# Autodesk Inventor assembly: ScreenHolderASM
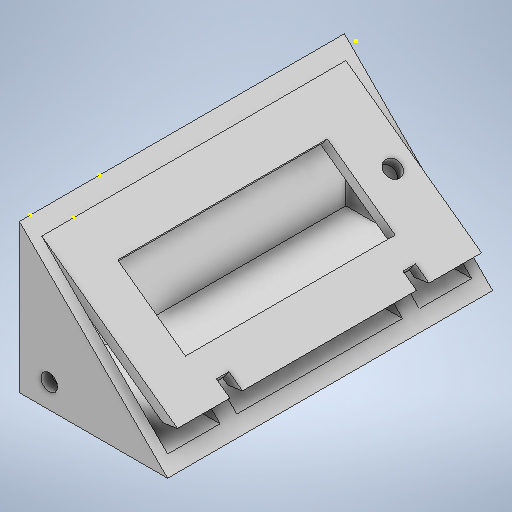
[picture p0: Inventor's stored thumbnail of the model, 512x512]
Saved by Autodesk Inventor 2025 (Build 290162000, 162)
## iProperties
Created: 2024-04-03
Part Number: ScreenHolderASM
Document SubType Name: Assembly
Designer: Daniel
Author: Daniel
## Documents named in this file (3)
- C:\Users\Daniel\Desktop\pmik_2024l_jd\mechanical\ScreenHolderASM.iam
- C:\Users\Daniel\Desktop\pmik_2024l_jd\mechanical\manuDisplayHolder.ipt
- C:\Users\Daniel\Desktop\pmik_2024l_jd\mechanical\menuDisplay.ipt
## Components (2 placed, 2 different names)
1. manuDisplayHolder:1 — Mate:1, Mate:2
2. menuDisplay:1 — Mate:1, Mate:2
## Relationships (2: Mate 2)
- Mate:1: manuDisplayHolder:1 ↔ menuDisplay:1
- Mate:2: manuDisplayHolder:1 ↔ menuDisplay:1
